# Autodesk Inventor assembly: 01EjectionPlate-Assembly
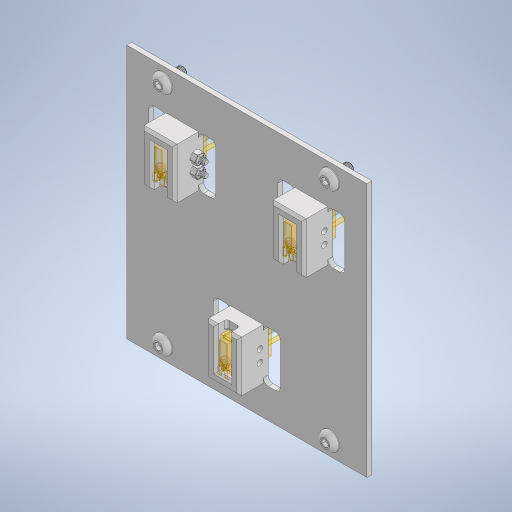
[picture p0: Inventor's stored thumbnail of the model, 512x512]
Saved by Autodesk Inventor 2023 (Build 270158000, 158)
## iProperties
Created: 2023-02-07
Part Number: 01EjectionPlate-Assembly
Document SubType Name: Assembly
Designer: 17038
Author: 17038
## Documents named in this file (6)
- C:\Users\17038\Desktop\02SheetMetalAseembly\EjectionPlateAssembly\01EjectionPlate-Assembly.iam
- C:\Users\17038\Desktop\02SheetMetalAseembly\EjectionPlateAssembly\01EjectionPlate.ipt
- C:\Users\17038\Desktop\CGA Sheetmetal\LimitSwitches\D2JW_01K1A1_MD_IGES\D2JW_01K1A1_MD.ipt
- C:\Users\17038\Desktop\CGA Sheetmetal\LimitSwitches\Hardware\92290A850_Super-Corrosion-Resistant 316 Stainless Steel Socket Head Screw.ipt
- C:\Users\17038\Desktop\CGA Sheetmetal\LimitSwitches\Locknut\93625A101_18-8 Stainless Steel Nylon-Insert Locknut.ipt
- C:\Users\17038\Desktop\CubeSat V4\Hardware\Ejection Plate\90943A114_Fine Thread 316 Stainless Steel Button Head Hex Drive Screw.ipt
## Components (12 placed, 5 different names)
1. 01EjectionPlate:1 — Mate:1, Flush:1, Mate:2, Mate:3, Mate:4, Mate:5, Mate:6, Mate:7, Mate:8, Mate:9, Mate:10, Mate:11, Flush:2, Mate:12, Mate:13, Flush:3, Mate:14
2. D2JW_01K1A1_MD:2 — Mate:13, Flush:3, Mate:14
3. D2JW_01K1A1_MD:3 — Mate:1, Flush:1, Mate:2
4. 92290A850_Super-Corrosion-Resistant 316 Stainless Steel Socket Head Screw:2 — Mate:4
5. 92290A850_Super-Corrosion-Resistant 316 Stainless Steel Socket Head Screw:3 — Mate:3
6. 93625A101_18-8 Stainless Steel Nylon-Insert Locknut:2 — Mate:6
7. 93625A101_18-8 Stainless Steel Nylon-Insert Locknut:3 — Mate:5
8. 90943A114_Fine Thread 316 Stainless Steel Button Head Hex Drive Screw:1 — Mate:7
9. 90943A114_Fine Thread 316 Stainless Steel Button Head Hex Drive Screw:2 — Mate:8
10. 90943A114_Fine Thread 316 Stainless Steel Button Head Hex Drive Screw:3 — Mate:9
11. 90943A114_Fine Thread 316 Stainless Steel Button Head Hex Drive Screw:4 — Mate:10
12. D2JW_01K1A1_MD:4 — Mate:11, Flush:2, Mate:12
## Relationships (17: Mate 14, Flush 3)
- Mate:1: 01EjectionPlate:1 ↔ D2JW_01K1A1_MD:3
- Flush:1: 01EjectionPlate:1 ↔ D2JW_01K1A1_MD:3
- Mate:2: 01EjectionPlate:1 ↔ D2JW_01K1A1_MD:3
- Mate:3: 01EjectionPlate:1 ↔ 92290A850_Super-Corrosion-Resistant 316 Stainless Steel Socket Head Screw:3
- Mate:4: 01EjectionPlate:1 ↔ 92290A850_Super-Corrosion-Resistant 316 Stainless Steel Socket Head Screw:2
- Mate:5: 01EjectionPlate:1 ↔ 93625A101_18-8 Stainless Steel Nylon-Insert Locknut:3
- Mate:6: 01EjectionPlate:1 ↔ 93625A101_18-8 Stainless Steel Nylon-Insert Locknut:2
- Mate:7: 01EjectionPlate:1 ↔ 90943A114_Fine Thread 316 Stainless Steel Button Head Hex Drive Screw:1
- Mate:8: 01EjectionPlate:1 ↔ 90943A114_Fine Thread 316 Stainless Steel Button Head Hex Drive Screw:2
- Mate:9: 01EjectionPlate:1 ↔ 90943A114_Fine Thread 316 Stainless Steel Button Head Hex Drive Screw:3
- Mate:10: 01EjectionPlate:1 ↔ 90943A114_Fine Thread 316 Stainless Steel Button Head Hex Drive Screw:4
- Mate:11: 01EjectionPlate:1 ↔ D2JW_01K1A1_MD:4
- Flush:2: 01EjectionPlate:1 ↔ D2JW_01K1A1_MD:4
- Mate:12: 01EjectionPlate:1 ↔ D2JW_01K1A1_MD:4
- Mate:13: 01EjectionPlate:1 ↔ D2JW_01K1A1_MD:2
- Flush:3: 01EjectionPlate:1 ↔ D2JW_01K1A1_MD:2
- Mate:14: 01EjectionPlate:1 ↔ D2JW_01K1A1_MD:2
